# Autodesk Inventor assembly: 組合1
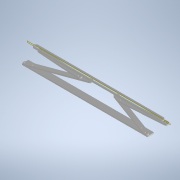
[picture p0: Inventor's stored thumbnail of the model, 180x180]
Saved by Autodesk Inventor 2022 (Build 260153000, 153)
## iProperties
Created: 2023-04-16
Part Number: 組合1
Document SubType Name: Assembly
Designer: JOU
Author: JOU
## Documents named in this file (5)
- C:\Users\JOU\Desktop\新增資料夾 (2)\組合1.iam
- C:\Users\JOU\Desktop\新增資料夾 (2)\零件1.ipt
- C:\Users\JOU\Desktop\新增資料夾 (2)\零件2.ipt
- C:\Users\JOU\Desktop\新增資料夾 (2)\零件3.ipt
- C:\Users\JOU\Desktop\新增資料夾 (2)\零件4.ipt
## Components (6 placed, 4 different names)
1. 零件1:1 — 插入:1, 插入:2, 角度:1
2. 零件2:1 — 插入:1, 插入:3, 貼合:2
3. 零件2:2 — 插入:2, 插入:4, 貼合:3
4. 零件3:1 — 插入:3, 貼合:1
5. 零件3:2 — 插入:4, 貼合:4, 貼合:5
6. 零件4:1 — 貼合:1, 貼合:2, 貼合:3, 貼合:4, 角度:1, 貼合:5
## Relationships (10: Mate 5, Insert 4, Angle 1)
- 插入:1 [Insert]: 零件1:1 ↔ 零件2:1
- 插入:2 [Insert]: 零件1:1 ↔ 零件2:2
- 插入:3 [Insert]: 零件2:1 ↔ 零件3:1
- 插入:4 [Insert]: 零件2:2 ↔ 零件3:2
- 貼合:1 [Mate]: 零件3:1 ↔ 零件4:1
- 貼合:2 [Mate]: 零件2:1 ↔ 零件4:1
- 貼合:3 [Mate]: 零件2:2 ↔ 零件4:1
- 貼合:4 [Mate]: 零件3:2 ↔ 零件4:1
- 角度:1 [Angle] (0 deg): 零件1:1 ↔ 零件4:1
- 貼合:5 [Mate]: 零件3:2 ↔ 零件4:1
